# Autodesk Inventor assembly: Gooseneck Model-1
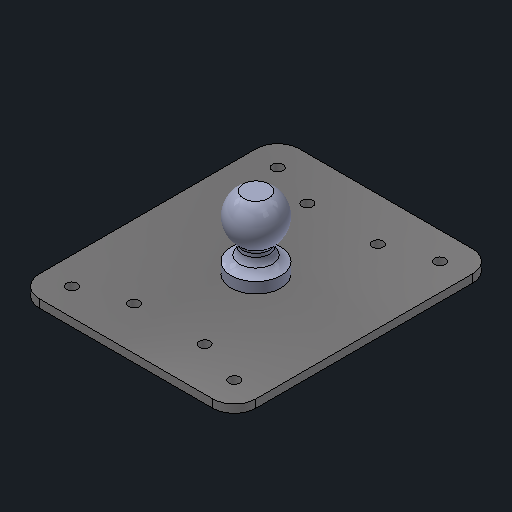
[picture p0: Inventor's stored thumbnail of the model, 512x512]
Saved by Autodesk Inventor 2025.1 (Build 291241000, 241)
## iProperties
Created: 2026-02-16
Part Number: Gooseneck Model-1
Document SubType Name: Assembly
Designer: Desktop -24
encoded128: ÌStandard (in)rÎ
Family: ASSEMBLY
Author: Desktop -24
## Documents named in this file (4)
- F:\OneDrive - nLeague Technologies Private Limited\Desktop\Sharath Chandra\Goose Neck\Gooseneck Model-2\Gooseneck Model-2.iam
- F:\OneDrive - nLeague Technologies Private Limited\Desktop\Sharath Chandra\Goose Neck\Gooseneck Model-2\Gooseneck Model-1 Ball.ipt
- F:\OneDrive - nLeague Technologies Private Limited\Desktop\Sharath Chandra\Goose Neck\Gooseneck Model-2\Gooseneck Model-1 Sheet-2.ipt
- F:\OneDrive - nLeague Technologies Private Limited\Desktop\Sharath Chandra\Goose Neck\Gooseneck Model-2\Gooseneck Model-2 Sheet-1.ipt
## Components (3 placed, 3 different names)
1. Gooseneck Model-2 Sheet-1:1 — Mate:1, Mate:2, Mate:3
2. Gooseneck Model-1 Ball:1 — Mate:1, Mate:2, Mate:4
3. Gooseneck Model-1 Sheet-2:1 — Mate:3, Mate:4
## Relationships (4: Mate 4)
- Mate:1: Gooseneck Model-2 Sheet-1:1 ↔ Gooseneck Model-1 Ball:1
- Mate:2 (12.7 mm): Gooseneck Model-2 Sheet-1:1 ↔ Gooseneck Model-1 Ball:1
- Mate:3: Gooseneck Model-2 Sheet-1:1 ↔ Gooseneck Model-1 Sheet-2:1
- Mate:4: Gooseneck Model-1 Ball:1 ↔ Gooseneck Model-1 Sheet-2:1
